# Autodesk Inventor assembly: BV-ASM-222-102
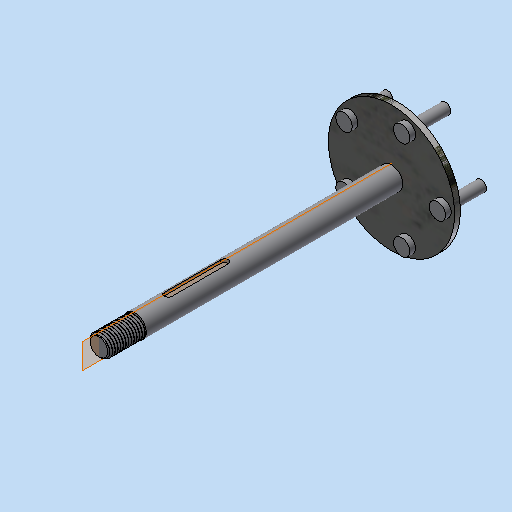
[picture p0: Inventor's stored thumbnail of the model, 512x512]
Saved by Autodesk Inventor 2025.3 (Build 293356030, 356C)
## iProperties
RuleStatus: InUse
Created: 2022-04-22
Part Number: BV-ASM-222-102
Document SubType Name: Assembly
Designer: josh Hofer
Description: WHEEL SHAFT ASSEMBLY
Mass: 905.145 g
Surface Area: 752.944 cm^2
Volume: 284.369 cm^3
Density: 3.183 g/cm^3
Author: josh Hofer
Revision Number: ANY
## iProperties of the stored document MemberDocs/xJbdrnimgPssx2lthSyk151gfPd
RuleStatus: InUse
Created: 2022-04-22
Part Number: BV-ASM-222-102
Document SubType Name: Assembly
Designer: josh Hofer
Description: WHEEL SHAFT ASSEMBLY
Mass: 905.145 g
Surface Area: 752.944 cm^2
Volume: 284.369 cm^3
Density: 3.183 g/cm^3
Author: josh Hofer
Revision Number: ANY
## Documents named in this file (7)
- R:\A1- Neuweg Design Data\OM Robotics\BASE VEHICLE DESIGN PROJECT\BV-ASM-222-102.iam
- R:\A1- Neuweg Design Data\OM Robotics\BASE VEHICLE DESIGN PROJECT\0222-113.ipt
- R:\A1- Neuweg Design Data\OM Robotics\BASE VEHICLE DESIGN PROJECT\0222-108.ipt
- R:\A1- Neuweg Design Data\OM Robotics\BASE VEHICLE DESIGN PROJECT\0222-107.ipt
- R:\A1- Neuweg Design Data\OM Robotics\BASE VEHICLE DESIGN PROJECT\96717A416.ipt
- R:\A1- Neuweg Design Data\OM Robotics\BASE VEHICLE DESIGN PROJECT\M12-1.50.ipt
- R:\A1- Neuweg Design Data\OM Robotics\BASE VEHICLE DESIGN PROJECT\4991T961.ipt
## Components (14 placed, 10 different names)
1. 0222-107 wheel shaft_344 — Insert:1, Mate:1, Mate:2, Mate:3, Flush:1, Flush:2
2. 0222-108 wheel hub adapter_345 — Insert:1, Insert:2, Insert:3, Insert:4, Insert:5, Insert:6, Insert:7, Mate:1, Insert:15, Insert:16, Insert:17, Insert:18, Insert:19, Insert:20
3. M12-1.50 wheel stud_346 — Insert:4
4. M12-1.50 wheel stud_347 — Insert:3
5. M12-1.50 wheel stud_348 — Insert:6
6. M12-1.50 wheel stud_349 — Insert:5
7. M12-1.50 wheel stud_350 — Insert:2, Insert:7
8. 4991T961:1 — Insert:17
9. 4991T961:2 — Insert:18
10. 4991T961:3 — Insert:19
11. 4991T961:4 — Insert:20
12. 4991T961:5 — Insert:16
13. 0222-113:1 — Insert:15
14. 96717A416:1 — Mate:2, Mate:3, Flush:1
## Relationships (18: Insert 13, Mate 3, Flush 2)
- Insert:1 (12.7 mm): 0222-107 wheel shaft_344 ↔ 0222-108 wheel hub adapter_345
- Insert:2: 0222-108 wheel hub adapter_345 ↔ M12-1.50 wheel stud_350
- Insert:3: 0222-108 wheel hub adapter_345 ↔ M12-1.50 wheel stud_347
- Insert:4: 0222-108 wheel hub adapter_345 ↔ M12-1.50 wheel stud_346
- Insert:5: 0222-108 wheel hub adapter_345 ↔ M12-1.50 wheel stud_349
- Insert:6: 0222-108 wheel hub adapter_345 ↔ M12-1.50 wheel stud_348
- Insert:7: 0222-108 wheel hub adapter_345 ↔ M12-1.50 wheel stud_350
- Mate:1: 0222-107 wheel shaft_344 ↔ 0222-108 wheel hub adapter_345
- Insert:15: 0222-108 wheel hub adapter_345 ↔ 0222-113:1
- Insert:16 (-4.8768 mm): 0222-108 wheel hub adapter_345 ↔ 4991T961:5
- Insert:17 (-4.8768 mm): 0222-108 wheel hub adapter_345 ↔ 4991T961:1
- Insert:18 (4.8768 mm): 0222-108 wheel hub adapter_345 ↔ 4991T961:2
- Insert:19 (4.8768 mm): 0222-108 wheel hub adapter_345 ↔ 4991T961:3
- Insert:20 (4.8768 mm): 0222-108 wheel hub adapter_345 ↔ 4991T961:4
- Mate:2: 0222-107 wheel shaft_344 ↔ 96717A416:1
- Mate:3: 0222-107 wheel shaft_344 ↔ 96717A416:1
- Flush:1 (-107.569 mm): 0222-107 wheel shaft_344 ↔ 96717A416:1
- Flush:2 (-107.5512 mm): 0222-107 wheel shaft_344
